# Autodesk Inventor assembly: L1 Gearbox Assembly_MIR
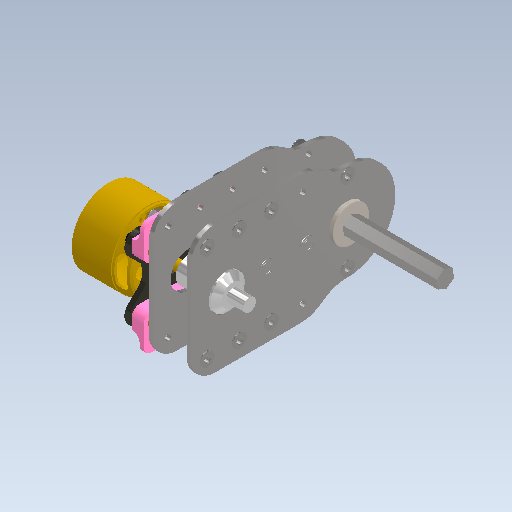
[picture p0: Inventor's stored thumbnail of the model, 512x512]
Saved by Autodesk Inventor 2023 (Build 270158000, 158)
## iProperties
Created: 2023-02-14
Part Number: L1 Gearbox Assembly_MIR
Document SubType Name: Assembly
Designer: Dave
Mass: 913.46 g
Surface Area: 1660.69 cm^2
Volume: 243.163 cm^3
Density: 3.75658 g/cm^3
Author: Dave
## Documents named in this file (15)
- C:\Users\Dave\Documents\GitHub\BehrendURCMechanical\CAD\Chassis V3\L1 Gearbox Assembly_MIR.iam
- C:\Users\Dave\Documents\GitHub\BehrendURCMechanical\CAD\Chassis\GearBox\Final Gears and Assemblies\CH-1-01-20T_Drive Gear_MIR1.ipt
- C:\Users\Dave\Documents\GitHub\BehrendURCMechanical\CAD\Chassis\GearBox\Final Gears and Assemblies\CH-1-01-60T_Output_MIR1.ipt
- C:\Users\Dave\Documents\GitHub\BehrendURCMechanical\CAD\Chassis\GearBox\Final Gears and Assemblies\CH-1-01-20T_Idler_MIR1.ipt
- C:\Users\Dave\Documents\GitHub\BehrendURCMechanical\CAD\Chassis\GearBox\Final Gears and Assemblies\CH-1-01-60T_Idler_MIR1.ipt
- C:\Users\Dave\Documents\GitHub\BehrendURCMechanical\CAD\Chassis\GearBox\Housing\CH-1-02-RearGearboxHousingMotorSide.ipt
- C:\Users\Dave\Documents\GitHub\BehrendURCMechanical\CAD\Chassis\GearBox\Drive Motor Shaft Coupler_MIR1.ipt
- C:\Users\Dave\Documents\GitHub\BehrendURCMechanical\CAD\Chassis V3\DriveMotorAssem\DriveMotorAssem_MIR.iam
- C:\Users\Dave\Documents\GitHub\BehrendURCMechanical\CAD\Chassis\GearBox\Ch-1-01-0.5x4.5HexShaft_MIR1.ipt
- C:\Users\Dave\Documents\GitHub\BehrendURCMechanical\CAD\Chassis\GearBox\CH-1-01-0.25x1.875SmoothShaft_MIR1.ipt
- C:\Users\Dave\Documents\GitHub\BehrendURCMechanical\CAD\Chassis\GearBox\CH-1-01-0.5HexBearing_MIR1.ipt
- C:\Users\Dave\Documents\GitHub\BehrendURCMechanical\CAD\Chassis\GearBox\CH-1-01-0.25IDSmoothBoreBearing_MIR1.ipt
- C:\Users\Dave\Downloads\91831A011_18-8 Stainless Steel Nylon-Insert Locknut (1)_MIR.ipt
- C:\Users\Dave\Documents\GitHub\BehrendURCMechanical\CAD\Chassis V3\90107A011_316 Stainless Steel Washer_MIR.ipt
- C:\Users\Dave\Documents\GitHub\BehrendURCMechanical\CAD\Chassis V3\L1Plate_MIR.ipt
## Components (45 placed, 14 different names)
1. CH-1-01-20T_Drive Gear_MIR1:1 — Insert:16
2. CH-1-01-60T_Output_MIR1:1 — Flush:6, Mate:17
3. CH-1-01-20T_Idler_MIR1:1 — Flush:5, Mate:21
4. CH-1-01-60T_Idler_MIR1:1 — Flush:5, Mate:19, Mate:20, Mate:18
5. CH-1-01-20T_Idler_MIR1:2 — Flush:6, Mate:19, Mate:22
6. CH-1-01-60T_Idler_MIR1:2 — Mate:11, Mate:10
7. CH-1-02-RearGearboxHousingMotorSide:1
8. CH-1-02-RearGearboxHousingMotorSide:2
9. Drive Motor Shaft Coupler_MIR1:1 — Insert:16, Mate:27, Mate:32, Mate:31
10. DriveMotorAssem_MIR:1 [sub-assembly] — Mate:27, Insert:61, Insert:60, Insert:59, Insert:67, Insert:68, Insert:69, Angle:2, Insert:66
11. Ch-1-01-0.5x4.5HexShaft_MIR1:1 — Flush:8, Mate:9, Mate:8
12. CH-1-01-0.25x1.875SmoothShaft_MIR1:1 — Insert:13
13. CH-1-01-0.25x1.875SmoothShaft_MIR1:2 — Insert:12, Flush:4
14. CH-1-01-0.5HexBearing_MIR1:1 — Flush:8, Mate:17
15. CH-1-01-0.5HexBearing_MIR1:2 — Mate:9, Mate:8, Mate:29, Mate:30
16. CH-1-01-0.25IDSmoothBoreBearing_MIR1:1 — Insert:12
17. CH-1-01-0.25IDSmoothBoreBearing_MIR1:2 — Mate:11, Insert:13
18. CH-1-01-0.25IDSmoothBoreBearing_MIR1:3 — Mate:22, Mate:20, Mate:18, Flush:4
19. CH-1-01-0.25IDSmoothBoreBearing_MIR1:4 — Mate:21, Mate:10
20. 91831A011_18-8 Stainless Steel Nylon-Insert Locknut (1)_MIR:1 — Insert:85
21. 91831A011_18-8 Stainless Steel Nylon-Insert Locknut (1)_MIR:2 — Insert:84
22. 91831A011_18-8 Stainless Steel Nylon-Insert Locknut (1)_MIR:3 — Insert:83
23. 91831A011_18-8 Stainless Steel Nylon-Insert Locknut (1)_MIR:4 — Insert:82
24. 91831A011_18-8 Stainless Steel Nylon-Insert Locknut (1)_MIR:5 — Insert:80
25. 91831A011_18-8 Stainless Steel Nylon-Insert Locknut (1)_MIR:6 — Insert:79
26. 91831A011_18-8 Stainless Steel Nylon-Insert Locknut (1)_MIR:7 — Insert:81
27. 91831A011_18-8 Stainless Steel Nylon-Insert Locknut (1)_MIR:8 — Insert:78
28. 90107A011_316 Stainless Steel Washer_MIR:1 — Insert:82, Insert:61
29. 90107A011_316 Stainless Steel Washer_MIR:2
30. 90107A011_316 Stainless Steel Washer_MIR:3
31. 90107A011_316 Stainless Steel Washer_MIR:4 — Insert:83, Insert:60
32. 90107A011_316 Stainless Steel Washer_MIR:5
33. 90107A011_316 Stainless Steel Washer_MIR:6 — Insert:84, Insert:59
34. 90107A011_316 Stainless Steel Washer_MIR:7 — Insert:53
35. 90107A011_316 Stainless Steel Washer_MIR:8 — Insert:85, Insert:51
36. 90107A011_316 Stainless Steel Washer_MIR:9 — Insert:57
37. 90107A011_316 Stainless Steel Washer_MIR:10 — Insert:78, Insert:55
38. 90107A011_316 Stainless Steel Washer_MIR:11
39. 90107A011_316 Stainless Steel Washer_MIR:12 — Insert:79, Insert:67
40. 90107A011_316 Stainless Steel Washer_MIR:13
41. 90107A011_316 Stainless Steel Washer_MIR:14 — Insert:80, Insert:68
42. 90107A011_316 Stainless Steel Washer_MIR:15
43. 90107A011_316 Stainless Steel Washer_MIR:16 — Insert:81, Insert:69
44. L1Plate_MIR:1 — Mate:32, Insert:57, Insert:53, Mate:29
45. L1Plate_MIR:2 — Angle:2, Insert:66, Insert:55, Insert:51, Mate:31, Mate:30
## Relationships (42: Insert 22, Mate 15, Flush 4, Angle 1)
- Flush:5: CH-1-01-20T_Idler_MIR1:1 ↔ CH-1-01-60T_Idler_MIR1:1
- Flush:6: CH-1-01-60T_Output_MIR1:1 ↔ CH-1-01-20T_Idler_MIR1:2
- Mate:19: CH-1-01-60T_Idler_MIR1:1 ↔ CH-1-01-20T_Idler_MIR1:2
- Insert:16: CH-1-01-20T_Drive Gear_MIR1:1 ↔ Drive Motor Shaft Coupler_MIR1:1
- Flush:8: Ch-1-01-0.5x4.5HexShaft_MIR1:1 ↔ CH-1-01-0.5HexBearing_MIR1:1
- Mate:17: CH-1-01-60T_Output_MIR1:1 ↔ CH-1-01-0.5HexBearing_MIR1:1
- Mate:9: Ch-1-01-0.5x4.5HexShaft_MIR1:1 ↔ CH-1-01-0.5HexBearing_MIR1:2
- Mate:8: Ch-1-01-0.5x4.5HexShaft_MIR1:1 ↔ CH-1-01-0.5HexBearing_MIR1:2
- Insert:12: CH-1-01-0.25x1.875SmoothShaft_MIR1:2 ↔ CH-1-01-0.25IDSmoothBoreBearing_MIR1:1
- Mate:11: CH-1-01-60T_Idler_MIR1:2 ↔ CH-1-01-0.25IDSmoothBoreBearing_MIR1:2
- Insert:13: CH-1-01-0.25x1.875SmoothShaft_MIR1:1 ↔ CH-1-01-0.25IDSmoothBoreBearing_MIR1:2
- Mate:22: CH-1-01-20T_Idler_MIR1:2 ↔ CH-1-01-0.25IDSmoothBoreBearing_MIR1:3
- Mate:20: CH-1-01-60T_Idler_MIR1:1 ↔ CH-1-01-0.25IDSmoothBoreBearing_MIR1:3
- Mate:18: CH-1-01-60T_Idler_MIR1:1 ↔ CH-1-01-0.25IDSmoothBoreBearing_MIR1:3
- Flush:4: CH-1-01-0.25x1.875SmoothShaft_MIR1:2 ↔ CH-1-01-0.25IDSmoothBoreBearing_MIR1:3
- Mate:21: CH-1-01-20T_Idler_MIR1:1 ↔ CH-1-01-0.25IDSmoothBoreBearing_MIR1:4
- Mate:10: CH-1-01-60T_Idler_MIR1:2 ↔ CH-1-01-0.25IDSmoothBoreBearing_MIR1:4
- Mate:27: Drive Motor Shaft Coupler_MIR1:1 ↔ DriveMotorAssem_MIR:1
- Insert:82: 91831A011_18-8 Stainless Steel Nylon-Insert Locknut (1)_MIR:4 ↔ 90107A011_316 Stainless Steel Washer_MIR:1
- Insert:61: DriveMotorAssem_MIR:1 ↔ 90107A011_316 Stainless Steel Washer_MIR:1
- Insert:83: 91831A011_18-8 Stainless Steel Nylon-Insert Locknut (1)_MIR:3 ↔ 90107A011_316 Stainless Steel Washer_MIR:4
- Insert:60: DriveMotorAssem_MIR:1 ↔ 90107A011_316 Stainless Steel Washer_MIR:4
- Insert:84: 91831A011_18-8 Stainless Steel Nylon-Insert Locknut (1)_MIR:2 ↔ 90107A011_316 Stainless Steel Washer_MIR:6
- Insert:59: DriveMotorAssem_MIR:1 ↔ 90107A011_316 Stainless Steel Washer_MIR:6
- Insert:85: 91831A011_18-8 Stainless Steel Nylon-Insert Locknut (1)_MIR:1 ↔ 90107A011_316 Stainless Steel Washer_MIR:8
- Insert:78: 91831A011_18-8 Stainless Steel Nylon-Insert Locknut (1)_MIR:8 ↔ 90107A011_316 Stainless Steel Washer_MIR:10
- Insert:79: 91831A011_18-8 Stainless Steel Nylon-Insert Locknut (1)_MIR:6 ↔ 90107A011_316 Stainless Steel Washer_MIR:12
- Insert:67: DriveMotorAssem_MIR:1 ↔ 90107A011_316 Stainless Steel Washer_MIR:12
- Insert:80: 91831A011_18-8 Stainless Steel Nylon-Insert Locknut (1)_MIR:5 ↔ 90107A011_316 Stainless Steel Washer_MIR:14
- Insert:68: DriveMotorAssem_MIR:1 ↔ 90107A011_316 Stainless Steel Washer_MIR:14
- Insert:81: 91831A011_18-8 Stainless Steel Nylon-Insert Locknut (1)_MIR:7 ↔ 90107A011_316 Stainless Steel Washer_MIR:16
- Insert:69: DriveMotorAssem_MIR:1 ↔ 90107A011_316 Stainless Steel Washer_MIR:16
- Mate:32: Drive Motor Shaft Coupler_MIR1:1 ↔ L1Plate_MIR:1
- Insert:57: 90107A011_316 Stainless Steel Washer_MIR:9 ↔ L1Plate_MIR:1
- Insert:53: 90107A011_316 Stainless Steel Washer_MIR:7 ↔ L1Plate_MIR:1
- Mate:29: CH-1-01-0.5HexBearing_MIR1:2 ↔ L1Plate_MIR:1
- Angle:2 (0 deg): DriveMotorAssem_MIR:1 ↔ L1Plate_MIR:2
- Insert:66: DriveMotorAssem_MIR:1 ↔ L1Plate_MIR:2
- Insert:55: 90107A011_316 Stainless Steel Washer_MIR:10 ↔ L1Plate_MIR:2
- Insert:51: 90107A011_316 Stainless Steel Washer_MIR:8 ↔ L1Plate_MIR:2
- Mate:31: Drive Motor Shaft Coupler_MIR1:1 ↔ L1Plate_MIR:2
- Mate:30: CH-1-01-0.5HexBearing_MIR1:2 ↔ L1Plate_MIR:2
